# Autodesk Inventor assembly: Final
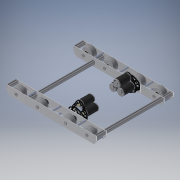
[picture p0: Inventor's stored thumbnail of the model, 180x180]
Saved by Autodesk Inventor 2016 (Build 200138000, 138)
## iProperties
Created: 2017-01-19
Part Number: Final
Document SubType Name: Assembly
Designer: Kyle
Author: Kyle
## Documents named in this file (9)
- E:\1073CAD\Robot2017\DriveTrain\Final.iam
- E:\1073CAD\Robot2017\DriveTrain\OutsidePlate.ipt
- E:\1073CAD\Robot2017\DriveTrain\Individual Parts\Mock 8020 28.25in.ipt
- E:\1073CAD\Robot2017\DriveTrain\InsidePlate.ipt
- E:\1073CAD\Robot2017\DriveTrain\Individual Parts\3.625Churro.ipt
- E:\1073CAD\Robot2017\DriveTrain\Individual Parts\SinglePulley.iam
- E:\1073CAD\Robot2017\DriveTrain\Individual Parts\DoublePulley.iam
- E:\1073CAD\Robot2017\DriveTrain\Individual Parts\DoublePulleyGearbox.iam
- E:\1073CAD\Robot2017\DriveTrain\Individual Parts\Mock 8020 3.375in.ipt
## Components (32 placed, 8 different names)
1. OutsidePlate:1 — Mate:1, Mate:2, Flush:1, Flush:2, Mate:3, Flush:3, Flush:4, Mate:5, Mate:6, Mate:7, Mate:8, Mate:9, Mate:10, Mate:11, Mate:12, Mate:29, Mate:30, Mate:31, Mate:32, Mate:33, Mate:34, Mate:37, Mate:38, Mate:43
2. Mock 8020 28.25in:1 — Mate:2, Flush:1, Flush:2, Mate:14
3. Mock 8020 28.25in:2 — Mate:1, Mate:3
4. InsidePlate:1 — Flush:3, Flush:4, Mate:13, Mate:42, Flush:9, Flush:10
5. 3.625Churro:1 — Mate:11
6. 3.625Churro:2 — Mate:10, Mate:13
7. 3.625Churro:3 — Mate:12
8. 3.625Churro:4 — Mate:9
9. 3.625Churro:5 — Mate:7
10. 3.625Churro:6 — Mate:8
11. 3.625Churro:7 — Mate:6
12. 3.625Churro:9 — Mate:5
13. OutsidePlate:2 — Mate:14, Mate:15, Mate:16, Mate:17, Mate:18, Mate:19, Mate:20, Mate:21, Mate:22, Flush:5, Flush:6, Mate:35, Mate:36, Mate:39, Mate:40
14. 3.625Churro:10 — Mate:15
15. 3.625Churro:11 — Mate:16
16. 3.625Churro:12 — Mate:17
17. 3.625Churro:13 — Mate:18
18. 3.625Churro:14 — Mate:19, Mate:24
19. 3.625Churro:15 — Mate:21
20. 3.625Churro:16 — Mate:20
21. 3.625Churro:18 — Mate:22
22. InsidePlate:2 — Flush:5, Flush:6, Mate:24, Mate:25, Mate:26, Mate:27, Mate:28, Mate:41, Mate:44, Flush:7, Flush:8
23. SinglePulley:1 [sub-assembly] — Mate:31, Mate:32
24. SinglePulley:2 [sub-assembly] — Mate:29, Mate:30
25. SinglePulley:3 [sub-assembly] — Mate:25, Mate:26
26. SinglePulley:4 [sub-assembly] — Mate:27, Mate:28
27. DoublePulley:1 [sub-assembly] — Mate:33, Mate:34
28. DoublePulley:2 [sub-assembly] — Mate:35, Mate:36
29. DoublePulleyGearbox:1 [sub-assembly] — Mate:37, Mate:38, Mate:42
30. DoublePulleyGearbox:2 [sub-assembly] — Mate:39, Mate:40, Mate:41
31. Mock 8020 3.375in:1 — Mate:43, Flush:9, Flush:10
32. Mock 8020 3.375in:2 — Mate:44, Flush:7, Flush:8
## Relationships (52: Mate 42, Flush 10)
- Mate:1: OutsidePlate:1 ↔ Mock 8020 28.25in:2
- Mate:2: OutsidePlate:1 ↔ Mock 8020 28.25in:1
- Flush:1 (6.35 mm): OutsidePlate:1 ↔ Mock 8020 28.25in:1
- Flush:2 (6.35 mm): OutsidePlate:1 ↔ Mock 8020 28.25in:1
- Mate:3: OutsidePlate:1 ↔ Mock 8020 28.25in:2
- Flush:3: OutsidePlate:1 ↔ InsidePlate:1
- Flush:4: OutsidePlate:1 ↔ InsidePlate:1
- Mate:5: OutsidePlate:1 ↔ 3.625Churro:9
- Mate:6: OutsidePlate:1 ↔ 3.625Churro:7
- Mate:7: OutsidePlate:1 ↔ 3.625Churro:5
- Mate:8: OutsidePlate:1 ↔ 3.625Churro:6
- Mate:9: OutsidePlate:1 ↔ 3.625Churro:4
- Mate:10: OutsidePlate:1 ↔ 3.625Churro:2
- Mate:11: OutsidePlate:1 ↔ 3.625Churro:1
- Mate:12: OutsidePlate:1 ↔ 3.625Churro:3
- Mate:13: InsidePlate:1 ↔ 3.625Churro:2
- Mate:14: Mock 8020 28.25in:1 ↔ OutsidePlate:2
- Mate:15: OutsidePlate:2 ↔ 3.625Churro:10
- Mate:16: OutsidePlate:2 ↔ 3.625Churro:11
- Mate:17: OutsidePlate:2 ↔ 3.625Churro:12
- Mate:18: OutsidePlate:2 ↔ 3.625Churro:13
- Mate:19: OutsidePlate:2 ↔ 3.625Churro:14
- Mate:20: OutsidePlate:2 ↔ 3.625Churro:16
- Mate:21: OutsidePlate:2 ↔ 3.625Churro:15
- Mate:22: OutsidePlate:2 ↔ 3.625Churro:18
- Flush:5: OutsidePlate:2 ↔ InsidePlate:2
- Flush:6: OutsidePlate:2 ↔ InsidePlate:2
- Mate:24: 3.625Churro:14 ↔ InsidePlate:2
- Mate:25: InsidePlate:2 ↔ SinglePulley:3
- Mate:26: InsidePlate:2 ↔ SinglePulley:3
- Mate:27: InsidePlate:2 ↔ SinglePulley:4
- Mate:28: InsidePlate:2 ↔ SinglePulley:4
- Mate:29: OutsidePlate:1 ↔ SinglePulley:2
- Mate:30: OutsidePlate:1 ↔ SinglePulley:2
- Mate:31: OutsidePlate:1 ↔ SinglePulley:1
- Mate:32: OutsidePlate:1 ↔ SinglePulley:1
- Mate:33: OutsidePlate:1 ↔ DoublePulley:1
- Mate:34: OutsidePlate:1 ↔ DoublePulley:1
- Mate:35: OutsidePlate:2 ↔ DoublePulley:2
- Mate:36: OutsidePlate:2 ↔ DoublePulley:2
- Mate:37: OutsidePlate:1 ↔ DoublePulleyGearbox:1
- Mate:38: OutsidePlate:1 ↔ DoublePulleyGearbox:1
- Mate:39: OutsidePlate:2 ↔ DoublePulleyGearbox:2
- Mate:40: OutsidePlate:2 ↔ DoublePulleyGearbox:2
- Mate:41: InsidePlate:2 ↔ DoublePulleyGearbox:2
- Mate:42: InsidePlate:1 ↔ DoublePulleyGearbox:1
- Mate:43: OutsidePlate:1 ↔ Mock 8020 3.375in:1
- Mate:44: InsidePlate:2 ↔ Mock 8020 3.375in:2
- Flush:7: InsidePlate:2 ↔ Mock 8020 3.375in:2
- Flush:8: InsidePlate:2 ↔ Mock 8020 3.375in:2
- Flush:9: InsidePlate:1 ↔ Mock 8020 3.375in:1
- Flush:10: InsidePlate:1 ↔ Mock 8020 3.375in:1
